# Autodesk Inventor assembly: MINI OFFSET
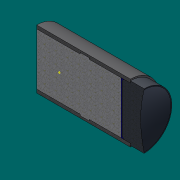
[picture p0: Inventor's stored thumbnail of the model, 180x180]
Saved by Autodesk Inventor 2011 SP1 (Build 150282100, 282)
## iProperties
Created: 2009-08-11
Part Number: MINI OFFSET
Document SubType Name: Assembly
Designer: bjones
MaterialNote: SEE BILL OF MATERIAL
Author: bjones
## Documents named in this file (5)
- G:\Engineering\Design\Brandon's work\Projects\2011 IVEC\Mike\MINI OFF SET\MINI OFFSET.IAM
- G:\Engineering\Design\Brandon's work\Projects\2011 IVEC\Mike\MINI\MINI BODY.ipt
- G:\Engineering\Design\Brandon's work\Projects\2011 IVEC\Mike\MINI\MINI CATHODE.ipt
- G:\Engineering\Design\Brandon's work\Projects\2011 IVEC\Mike\MINI\POTTING.ipt
- G:\Engineering\Design\Brandon's work\Projects\2011 IVEC\Mike\MINI\BRAZE COAT.ipt
## Components (4 placed, 4 different names)
1. MINI BODY:1 — Mate:1, Mate:2, Mate:3
2. MINI CATHODE:1 — Mate:3, Mate:4, Mate:7
3. POTTING:1 — Mate:5, Mate:8
4. BRAZE COAT:1 — Mate:6, Mate:7, Flush:1, Mate:8
## Relationships (9: Mate 8, Flush 1)
- Mate:1: MINI BODY:1
- Mate:2: MINI BODY:1
- Mate:3: MINI BODY:1 ↔ MINI CATHODE:1
- Mate:4: MINI CATHODE:1
- Mate:5: POTTING:1
- Mate:6: BRAZE COAT:1
- Mate:7: MINI CATHODE:1 ↔ BRAZE COAT:1
- Flush:1: BRAZE COAT:1
- Mate:8: POTTING:1 ↔ BRAZE COAT:1
